# Autodesk Inventor assembly: SCSWA8-8
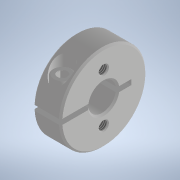
[picture p0: Inventor's stored thumbnail of the model, 180x180]
Saved by Autodesk Inventor 2021 (Build 250183000, 183)
## iProperties
Category: PARTsolutions
Company: MISUMI
Created: 2025-04-08
Part Number: SCSWA8-8
Catalog Web Link: www.cadenas.de
Description: SCSW, PSCSW, SSCSW, SCSWA, SCSWAW-Set Collars - Slit 2 Hole/2 Tap - Standard Type - 2 Tap Type
Vendor: MISUMI
Document SubType Name: Assembly
Designer: psAdmin
Manufacturer: MISUMI
Mass: 3.19807 g
Surface Area: 22.4596 cm^2
Volume: 3.19807 cm^3
Density: 1 g/cm^3
Title: SCSWA8-8
Author: Cadenas PARTsolutions
Comments: Set Collars - Slit 2 Hole/2 Tap - Standard Type - 2 Tap Type
PSOL_IDENT_0: {$CADENAS_DATA/23d-libs/misumi/metric/03_set_collars/scsw_asmtab.prj},208 {VTYP=3D},{STYP=ASSTAB},{N
PSOL_IDENT_1: B=SCSWA8-8},{LINA=SCSWA8-8},{NN=SCSW, PSCSW, SSCSW, SCSWA, SCSWAW},{DATE=29.11.2024 04:05:21},{GEOMD
PSOL_IDENT_2: ATE=15.09.2021 06:02:54},{VERSION=},{LINEID=50},{WBVAR=MAT,ST,BS},{WBNUMERIC=BS}  {NB=SCSWA8-8},{LIN
PSOL_IDENT_3: A=SCSWA8-8},{KT=DUMMY},{PN=SCSWA8-8},{TYPE=SCSWA},{MAT=2017},{MATA='1045','S45C Equivalent','304','S
PSOL_IDENT_4: US304 Equivalent','2017','2017 Aluminum Alloy'},{ST=-},{AC=Hexagon Socket Head Set Screw 1 Pc. (304
PSOL_IDENT_5: Stainless Steel) },{D=8},{BS=8},{B1=8,10,12},{D1=25},{M=M3},{THMD=3},{THDMIN=2.459},{ST0='-','-','Cl
PSOL_IDENT_6: ear Anodize','Clear Anodize'},{DD=3.4},{R=3.00},{W=1.5},{X=8.0},{Y=5.0},{Z=7~9},{S=3.5},{P=14},{C=0.
PSOL_IDENT_7: 5},{L=10},{M1=M3},{ZZ=8},{THMD1=3},{THDMIN1=2.459},{PPATH=scsw_templ.prj}
NB: SCSWA8-8
NN: SCSW, PSCSW, SSCSW, SCSWA, SCSWAW
NT: Set Collars - Slit 2 Hole/2 Tap - Standard Type - 2 Tap Type
NBSYN: $PN.
LINA: SCSWA8-8
CATALOG: Misumi
PN: SCSWA8-8
MAT: 2017 Aluminum Alloy
ST: -
AC: Hexagon Socket Head Set Screw 1 Pc. (304 Stainless Steel)
D: 8
BS: 8
D1: 25
M: M3
DD: 3.4
R: 3
W: 1.5
X: 8
Y: 5
Z: 7~9
S: 3.5
P: 14
M1: M3
SUPPLIER: MISUMI
ARTICLENO: SCSWA8-8
BOMINFO: SCSWA8-8
CREATOR: CADENAS GmbH
## Documents named in this file (3)
- e:\temp\worker_COMMON_17\temp\tmp_5832_32_x10nv\format_0\SCSWA8-8.iam
- e:\temp\worker_COMMON_17\temp\tmp_5832_32_x10nv\format_0\SCSWA8-8b.ipt
- e:\temp\worker_COMMON_17\temp\tmp_5832_32_x10nv\format_0\Slotted head cap screw ISO 4762 - M3x10.ipt
## Components (2 placed, 2 different names)
1. SCSWA8-8b:1 — body_screw_Z@1 <-> IP1_Z@2
2. Slotted head cap screw ISO 4762 - M3x10:1 — body_screw_Z@1 <-> IP1_Z@2
## Relationships (1: Mate 1)
- body_screw_Z@1 <-> IP1_Z@2 [Mate]: SCSWA8-8b:1 ↔ Slotted head cap screw ISO 4762 - M3x10:1
